# Autodesk Inventor assembly: Assembly1
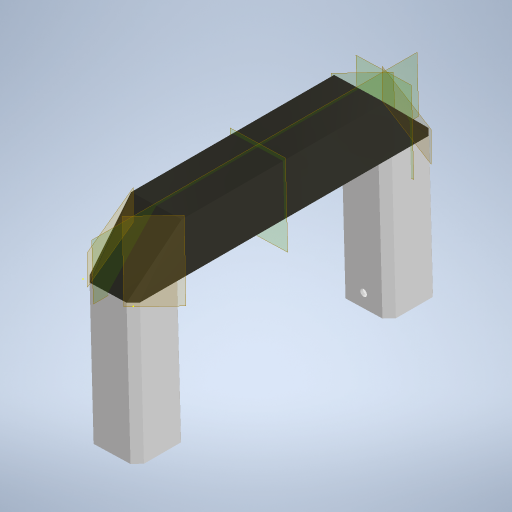
[picture p0: Inventor's stored thumbnail of the model, 512x512]
Saved by Autodesk Inventor 2024 (Build 280153000, 153)
## iProperties
Created: 2024-04-21
Part Number: Assembly1
Document SubType Name: Assembly
Designer: kamil
Author: kamil
## Documents named in this file (4)
- D:\Projects\Robotics\Linefollower_competition_gate\Assembly1.iam
- D:\Projects\Robotics\Linefollower_competition_gate\connector_part.ipt
- D:\Projects\Robotics\Linefollower_competition_gate\detector_leg.ipt
- D:\Projects\Robotics\Linefollower_competition_gate\laser_leg.ipt
## Components (3 placed, 3 different names)
1. connector_part:1 — Mate:2, Mate:3, Mate:4, Mate:5, Mate:6
2. detector_leg:1 — Mate:1, Mate:2, Mate:3, Mate:6
3. laser_leg:1 — Mate:1, Mate:4, Mate:5
## Relationships (6: Mate 6)
- Mate:1: detector_leg:1 ↔ laser_leg:1
- Mate:2: connector_part:1 ↔ detector_leg:1
- Mate:3: connector_part:1 ↔ detector_leg:1
- Mate:4: connector_part:1 ↔ laser_leg:1
- Mate:5: connector_part:1 ↔ laser_leg:1
- Mate:6: connector_part:1 ↔ detector_leg:1
